# Autodesk Inventor assembly: ClimbMechanism
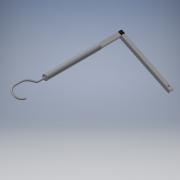
[picture p0: Inventor's stored thumbnail of the model, 180x180]
Saved by Autodesk Inventor 2017 (Build 210142000, 142)
## iProperties
Created: 2020-02-10
Part Number: ClimbMechanism
Document SubType Name: Assembly
Designer: S338674153
Author: S338674153
## Documents named in this file (7)
- \\ad.ocdsb.ca\studenthome\3\S338674153\FRC 2020\Modular Frame With 18in Brace\ClimbMechanism.iam
- \\ad.ocdsb.ca\studenthome\3\S338674153\FRC 2020\Modular Frame With 18in Brace\2nd arm.ipt
- \\ad.ocdsb.ca\studenthome\3\S338674153\FRC 2020\Modular Frame With 18in Brace\Cylinder 1.ipt
- \\ad.ocdsb.ca\studenthome\3\S338674153\FRC 2020\Modular Frame With 18in Brace\Cylinder Rod 1.ipt
- \\ad.ocdsb.ca\studenthome\3\S338674153\FRC 2020\Modular Frame With 18in Brace\Climb_Hook.ipt
- \\ad.ocdsb.ca\studenthome\3\S338674153\FRC 2020\Modular Frame With 18in Brace\90 joint piece.ipt
- \\ad.ocdsb.ca\studenthome\3\S338674153\FRC 2020\Modular Frame With 18in Brace\16 inch arm.ipt
## Components (6 placed, 6 different names)
1. 2nd arm:1 — Mate:3, Mate:4, Mate:7, Mate:8, Mate:9
2. Cylinder 1:1 — Mate:1, Mate:2, Mate:3, Mate:4
3. Cylinder Rod 1:1 — Mate:1, Mate:2, Mate:5, Mate:6
4. Climb_Hook:1 — Mate:5, Mate:6
5. 90 joint piece:1 — Mate:7, Mate:8, Mate:9, Mate:10, Mate:11, Mate:12
6. 16 inch arm:1 — Mate:10, Mate:11, Mate:12
## Relationships (12: Mate 12)
- Mate:1: Cylinder 1:1 ↔ Cylinder Rod 1:1
- Mate:2: Cylinder 1:1 ↔ Cylinder Rod 1:1
- Mate:3: 2nd arm:1 ↔ Cylinder 1:1
- Mate:4: 2nd arm:1 ↔ Cylinder 1:1
- Mate:5: Cylinder Rod 1:1 ↔ Climb_Hook:1
- Mate:6: Cylinder Rod 1:1 ↔ Climb_Hook:1
- Mate:7: 2nd arm:1 ↔ 90 joint piece:1
- Mate:8: 2nd arm:1 ↔ 90 joint piece:1
- Mate:9: 2nd arm:1 ↔ 90 joint piece:1
- Mate:10: 90 joint piece:1 ↔ 16 inch arm:1
- Mate:11: 90 joint piece:1 ↔ 16 inch arm:1
- Mate:12: 90 joint piece:1 ↔ 16 inch arm:1
